# Autodesk Inventor assembly: new collector mount
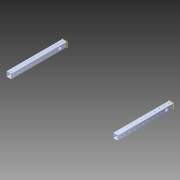
[picture p0: Inventor's stored thumbnail of the model, 180x180]
Saved by Autodesk Inventor 2014 SP1 (Build 180222100, 222)
## iProperties
Created: 2014-01-17
Part Number: new collector mount
Document SubType Name: Assembly
Designer: Arpan
Author: Arpan
## Documents named in this file (2)
- C:\Users\Arpan\Documents\GitHub\2014buildCAD\new collector mount\new collector mount.iam
- C:\Users\Arpan\Documents\GitHub\2014buildCAD\new collector mount\Vex Pro 1x1 rectangular tubing 9 in length.ipt
## Components (2 placed, 1 different names)
1. Vex Pro 1x1 rectangular tubing 9 in length:1 — Mate:1, Flush:1, Flush:2
2. Vex Pro 1x1 rectangular tubing 9 in length:2 — Mate:1, Flush:1, Flush:2
## Relationships (3: Flush 2, Mate 1)
- Mate:1 (558.8 mm): Vex Pro 1x1 rectangular tubing 9 in length:1 ↔ Vex Pro 1x1 rectangular tubing 9 in length:2
- Flush:1: Vex Pro 1x1 rectangular tubing 9 in length:1 ↔ Vex Pro 1x1 rectangular tubing 9 in length:2
- Flush:2: Vex Pro 1x1 rectangular tubing 9 in length:1 ↔ Vex Pro 1x1 rectangular tubing 9 in length:2
